# Autodesk Inventor assembly: Moving Carousel Section Assembly
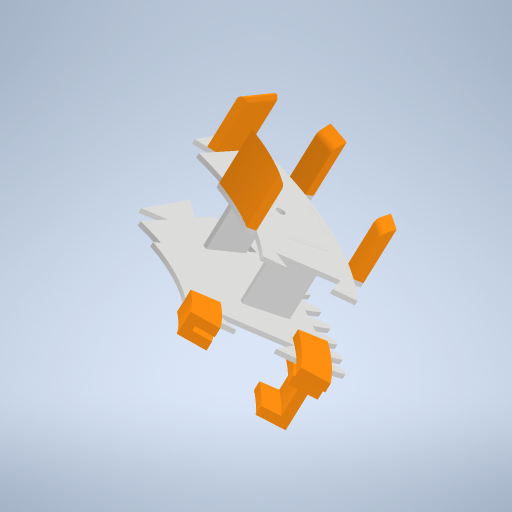
[picture p0: Inventor's stored thumbnail of the model, 512x512]
Saved by Autodesk Inventor 2023 (Build 270158000, 158)
## iProperties
Created: 2023-02-14
Part Number: Moving Carousel Section Assembly
Document SubType Name: Assembly
Designer: cheng
Author: cheng
## Documents named in this file (6)
- C:\Users\mihal\Desktop\4th Year Project\Final Assembly\Rotating Carousel\Moving Carousel Section Assembly.iam
- C:\Users\mihal\Desktop\4th Year Project\Final Assembly\Rotating Carousel\Rotating Carousel Geared Plate.ipt
- C:\Users\mihal\Desktop\4th Year Project\Final Assembly\Rotating Carousel\Rotating Carousel Wall.ipt
- C:\Users\mihal\Desktop\4th Year Project\Final Assembly\Rotating Carousel\Rotating Carousel Outer Clip.ipt
- C:\Users\mihal\Desktop\4th Year Project\Final Assembly\Rotating Carousel\Rotating Carousel Inner Clip.ipt
- C:\Users\mihal\Desktop\4th Year Project\Final Assembly\Rotating Carousel\Rotating Carousel Top Plate with Divider Walls.ipt
## Components (7 placed, 5 different names)
1. Rotating Carousel Wall:1 — Mate:3, Flush:2, Mate:4
2. Rotating Carousel Wall:2 — Flush:3, Mate:5, Mate:6, Mate:13, Flush:4, Mate:14
3. Rotating Carousel Wall:3 — Flush:1, Mate:1, Mate:2
4. Rotating Carousel Geared Plate:1 — Flush:1, Mate:1, Mate:2, Mate:3, Flush:2, Mate:4, Flush:3, Mate:5, Mate:6, Mate:7, Mate:8, Mate:9, Mate:10, Mate:11, Mate:12
5. Rotating Carousel Outer Clip:1 — Mate:7, Mate:8, Mate:9
6. Rotating Carousel Inner Clip:1 — Mate:10, Mate:11, Mate:12
7. Rotating Carousel Top Plate with Divider Walls:1 — Mate:13, Flush:4, Mate:14
## Relationships (18: Mate 14, Flush 4)
- Flush:1: Rotating Carousel Wall:3 ↔ Rotating Carousel Geared Plate:1
- Mate:1: Rotating Carousel Wall:3 ↔ Rotating Carousel Geared Plate:1
- Mate:2: Rotating Carousel Wall:3 ↔ Rotating Carousel Geared Plate:1
- Mate:3: Rotating Carousel Wall:1 ↔ Rotating Carousel Geared Plate:1
- Flush:2: Rotating Carousel Wall:1 ↔ Rotating Carousel Geared Plate:1
- Mate:4: Rotating Carousel Wall:1 ↔ Rotating Carousel Geared Plate:1
- Flush:3: Rotating Carousel Wall:2 ↔ Rotating Carousel Geared Plate:1
- Mate:5: Rotating Carousel Wall:2 ↔ Rotating Carousel Geared Plate:1
- Mate:6: Rotating Carousel Wall:2 ↔ Rotating Carousel Geared Plate:1
- Mate:7: Rotating Carousel Geared Plate:1 ↔ Rotating Carousel Outer Clip:1
- Mate:8: Rotating Carousel Geared Plate:1 ↔ Rotating Carousel Outer Clip:1
- Mate:9: Rotating Carousel Geared Plate:1 ↔ Rotating Carousel Outer Clip:1
- Mate:10: Rotating Carousel Geared Plate:1 ↔ Rotating Carousel Inner Clip:1
- Mate:11: Rotating Carousel Geared Plate:1 ↔ Rotating Carousel Inner Clip:1
- Mate:12: Rotating Carousel Geared Plate:1 ↔ Rotating Carousel Inner Clip:1
- Mate:13: Rotating Carousel Wall:2 ↔ Rotating Carousel Top Plate with Divider Walls:1
- Flush:4: Rotating Carousel Wall:2 ↔ Rotating Carousel Top Plate with Divider Walls:1
- Mate:14: Rotating Carousel Wall:2 ↔ Rotating Carousel Top Plate with Divider Walls:1
